# Autodesk Inventor assembly: Module_MFC
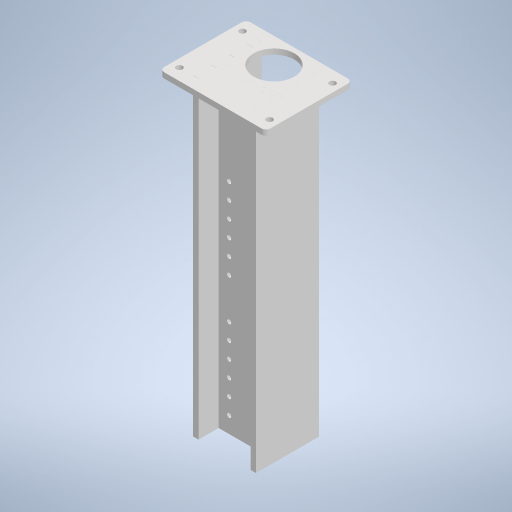
[picture p0: Inventor's stored thumbnail of the model, 512x512]
Saved by Autodesk Inventor 2023 (Build 270158000, 158)
## iProperties
Created: 2022-11-04
Part Number: Module_MFC
Document SubType Name: Assembly
Designer: incep
Author: incep
## Documents named in this file (4)
- C:\Users\incep\OneDrive\Desktop\Laser Cutter Things\ModularUhOhChair\Module_MFC.iam
- C:\Users\incep\OneDrive\Desktop\Laser Cutter Things\ModularUhOhChair\Module_base_MFC.ipt
- C:\Users\incep\OneDrive\Desktop\Laser Cutter Things\ModularUhOhChair\Module_supportX_MFC.ipt
- C:\Users\incep\OneDrive\Desktop\Laser Cutter Things\ModularUhOhChair\Module_supportZ_MFC.ipt
## Components (4 placed, 3 different names)
1. Module_base_MFC:1 — Flush:1, Mate:1, Flush:2, Flush:3, Flush:4
2. Module_supportX_MFC:1 — Mate:1, Flush:2, Mate:2, Mate:3
3. Module_supportZ_MFC:1 — Mate:2, Flush:3
4. Module_supportZ_MFC:2 — Mate:3, Flush:4
## Relationships (7: Flush 4, Mate 3)
- Flush:1: Module_base_MFC:1
- Mate:1: Module_base_MFC:1 ↔ Module_supportX_MFC:1
- Flush:2: Module_base_MFC:1 ↔ Module_supportX_MFC:1
- Mate:2: Module_supportX_MFC:1 ↔ Module_supportZ_MFC:1
- Flush:3: Module_base_MFC:1 ↔ Module_supportZ_MFC:1
- Mate:3: Module_supportX_MFC:1 ↔ Module_supportZ_MFC:2
- Flush:4: Module_base_MFC:1 ↔ Module_supportZ_MFC:2
